# Autodesk Inventor assembly: MicroD_FFC_Support
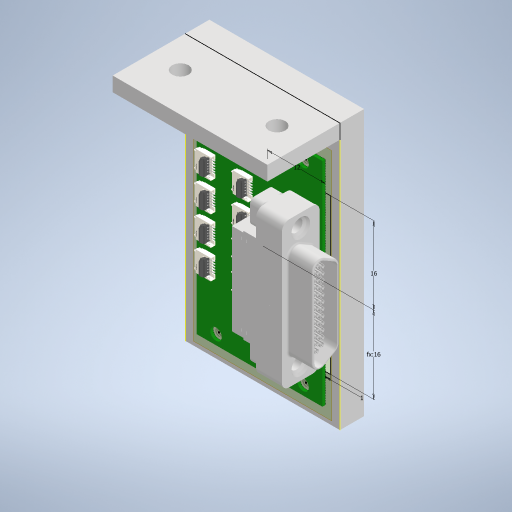
[picture p0: Inventor's stored thumbnail of the model, 512x512]
Saved by Autodesk Inventor 2024 (Build 280153000, 153)
## iProperties
Created: 2025-11-07
Part Number: MicroD_FFC_Support
Document SubType Name: Assembly
Designer: alexi
Author: alexi
## Documents named in this file (3)
- C:\Jeonghyun\SNU_GIT\QSTL_MicroDSUB_FFC\Support\MicroD_FFC_Support.iam
- C:\Jeonghyun\SNU_GIT\QSTL_MicroDSUB_FFC\Support\QSTL_MicroDSUB_FFC\QSTL_MicroDSUB_FFC.iam
- C:\Jeonghyun\SNU_GIT\QSTL_MicroDSUB_FFC\Support\Support.ipt
## Components (2 placed, 2 different names)
1. QSTL_MicroDSUB_FFC:1 [sub-assembly] — 플러쉬:1, 플러쉬:2
2. Support:1 — 플러쉬:1, 플러쉬:2
## Relationships (2: Flush 2)
- 플러쉬:1 [Flush]: QSTL_MicroDSUB_FFC:1 ↔ Support:1
- 플러쉬:2 [Flush]: QSTL_MicroDSUB_FFC:1 ↔ Support:1
